# Autodesk Inventor assembly: Mold Design1
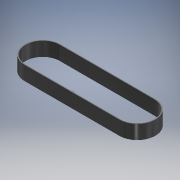
[picture p0: Inventor's stored thumbnail of the model, 180x180]
Saved by Autodesk Inventor 2018 (Build 220112000, 112)
## iProperties
Created: 2018-06-05
Part Number: Mold Design1
Document SubType Name: Assembly
Designer: P241310
Author: P241310
## Documents named in this file (3)
- C:\Users\P241310\Documents\GitHub\mecanum-cad\Mold Design1\Mold Design1.iam
- C:\Users\P241310\Documents\GitHub\mecanum-cad\Tooth1.ipt
- C:\Users\P241310\Documents\GitHub\mecanum-cad\Synchronous Belt1.ipt
## Components (3 placed, 2 different names)
1. Synchronous Belt:1 — Mate:1
2. Tooth1:1 — Mate:1
3. Tooth1:2
## Component patterns: (2 elements, first: Tooth1:1)
## Relationships (1: Mate 1)
- Mate:1: Synchronous Belt:1 ↔ Tooth1:1
